# Autodesk Inventor assembly: mabuchi 555+IG32
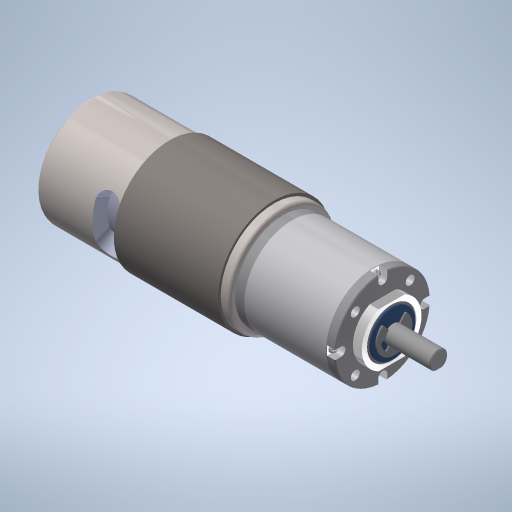
[picture p0: Inventor's stored thumbnail of the model, 512x512]
Saved by Autodesk Inventor 2023 (Build 270158000, 158)
## iProperties
Created: 2018-10-19
Part Number: mabuchi 555+IG32
Material: 一般
Document SubType Name: Assembly
Designer: shun
Author: shun
## Documents named in this file (3)
- C:\Users\blueh\OneDrive - Kyushu University\2023NHK_RR_2ndvid\000_parts_zegi\motor\mabuchi 555+IG32.iam
- C:\Users\blueh\Desktop\zip - コピー\Mabuchi 555.ipt
- C:\Users\blueh\Desktop\zip - コピー\IG-32_51以上.ipt
## Components (2 placed, 2 different names)
1. Mabuchi 555:1 — メイト:1, メイト:2, 角度:1
2. IG-32_51以上:1 — メイト:1, メイト:2, 角度:1
## Relationships (3: Mate 2, Angle 1)
- メイト:1 [Mate]: Mabuchi 555:1 ↔ IG-32_51以上:1
- メイト:2 [Mate]: Mabuchi 555:1 ↔ IG-32_51以上:1
- 角度:1 [Angle] (0 deg): Mabuchi 555:1 ↔ IG-32_51以上:1
